# Autodesk Inventor assembly: Assembly2
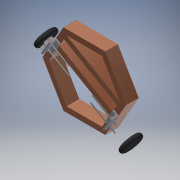
[picture p0: Inventor's stored thumbnail of the model, 180x180]
Saved by Autodesk Inventor 2017 (Build 210142000, 142)
## iProperties
Created: 2018-10-17
Part Number: Assembly2
Document SubType Name: Assembly
Designer: Administrator
Author: Administrator
## Documents named in this file (7)
- C:\Users\Administrator\Documents\GitHub\tr2\Base\Base.iam
- C:\Users\Administrator\Documents\GitHub\tr2\BA01.ipt
- C:\Users\Administrator\Documents\GitHub\tr2\BA02.ipt
- C:\Users\Administrator\Documents\GitHub\tr2\Scooter Wheel.ipt
- C:\Users\Administrator\Documents\GitHub\tr2\BA03.ipt
- C:\Users\Administrator\Documents\GitHub\tr2\8mm Shaft.ipt
- C:\Users\Administrator\Documents\GitHub\tr2\Base\Base\Design Accelerator\Spur Gears1.iam
## Components (17 placed, 6 different names)
1. BA01:1 — Mate:1, Flush:1, Mate:6, Mate:9, Flush:3, Mate:10
2. BA01:2 — Mate:2, Mate:4, Mate:5, Mate:7, Mate:8, Flush:2, Mate:17, Flush:7
3. BA01:3 — Mate:7, Mate:8, Flush:2
4. BA01:4 — Mate:11, Flush:4, Mate:12
5. BA01:5 — Mate:9, Flush:3, Mate:10, Mate:11, Flush:4, Mate:12, Mate:13, Flush:5, Mate:14, Flush:6, Mate:15, Mate:26, Flush:11
6. BA01:6 — Mate:1, Mate:2, Mate:4, Mate:5, Flush:1, Mate:6
7. BA02:1 — Mate:13, Flush:5, Mate:14, Mate:16, Flush:8, Flush:12
8. BA02:2 — Flush:6, Mate:15, Mate:16
9. BA03:1 — Mate:17, Flush:7, Flush:8, Mate:18, Mate:19, Mate:21, Mate:23
10. Scooter Wheel:1 — Mate:24, Mate:25, Flush:9
11. Scooter Wheel:2 — Mate:29
12. 8mm Shaft:1 — Mate:18, Mate:22, Mate:24, Flush:9
13. 8mm Shaft:2 — Mate:19, Mate:20, Flush:10
14. Spur Gears:1 [sub-assembly] — Mate:20, Mate:21, Mate:22, Mate:23, Mate:25, Flush:10
15. BA03:2 — Mate:26, Flush:11, Mate:27, Mate:28, Flush:12
16. 8mm Shaft:3 — Mate:28
17. 8mm Shaft:4 — Mate:27, Mate:29
## Relationships (40: Mate 28, Flush 12)
- Mate:1: BA01:1 ↔ BA01:6
- Mate:2: BA01:2 ↔ BA01:6
- Mate:4: BA01:2 ↔ BA01:6
- Mate:5: BA01:2 ↔ BA01:6
- Flush:1: BA01:1 ↔ BA01:6
- Mate:6: BA01:1 ↔ BA01:6
- Mate:7: BA01:2 ↔ BA01:3
- Mate:8: BA01:2 ↔ BA01:3
- Flush:2: BA01:2 ↔ BA01:3
- Mate:9: BA01:1 ↔ BA01:5
- Flush:3: BA01:1 ↔ BA01:5
- Mate:10: BA01:1 ↔ BA01:5
- Mate:11: BA01:4 ↔ BA01:5
- Flush:4: BA01:4 ↔ BA01:5
- Mate:12: BA01:4 ↔ BA01:5
- Mate:13: BA01:5 ↔ BA02:1
- Flush:5: BA01:5 ↔ BA02:1
- Mate:14: BA01:5 ↔ BA02:1
- Flush:6: BA01:5 ↔ BA02:2
- Mate:15: BA01:5 ↔ BA02:2
- Mate:16 (63.5 mm): BA02:1 ↔ BA02:2
- Mate:17: BA01:2 ↔ BA03:1
- Flush:7: BA01:2 ↔ BA03:1
- Flush:8 (81.025 mm): BA02:1 ↔ BA03:1
- Mate:18: BA03:1 ↔ 8mm Shaft:1
- Mate:19: BA03:1 ↔ 8mm Shaft:2
- Mate:20: 8mm Shaft:2 ↔ Spur Gears:1
- Mate:21: BA03:1 ↔ Spur Gears:1
- Mate:22: 8mm Shaft:1 ↔ Spur Gears:1
- Mate:23: BA03:1 ↔ Spur Gears:1
- Mate:24: Scooter Wheel:1 ↔ 8mm Shaft:1
- Mate:25: Scooter Wheel:1 ↔ Spur Gears:1
- Flush:9: Scooter Wheel:1 ↔ 8mm Shaft:1
- Flush:10: 8mm Shaft:2 ↔ Spur Gears:1
- Mate:26: BA01:5 ↔ BA03:2
- Flush:11: BA01:5 ↔ BA03:2
- Mate:27: BA03:2 ↔ 8mm Shaft:4
- Mate:28: BA03:2 ↔ 8mm Shaft:3
- Flush:12 (81.025 mm): BA02:1 ↔ BA03:2
- Mate:29: Scooter Wheel:2 ↔ 8mm Shaft:4
